# Autodesk Inventor assembly: sheetmetal_cnc
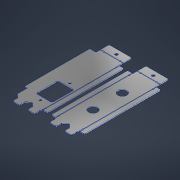
[picture p0: Inventor's stored thumbnail of the model, 180x180]
Saved by Autodesk Inventor 2022 (Build 260153000, 153)
## iProperties
Created: 2025-03-03
Part Number: sheetmetal_cnc
Document SubType Name: Assembly
Designer: gisen
Author: gisen
## Documents named in this file (3)
- C:\Users\gisen\Documents\CAD\inventor\git\eatx_case\eatx_slim\sheetmetal_cnc.iam
- C:\Users\gisen\Documents\CAD\inventor\git\eatx_case\eatx_slim\parts\power_ac_plate.ipt
- C:\Users\gisen\Documents\CAD\inventor\git\eatx_case\eatx_slim\parts\power_sw_plate.ipt
## Components (2 placed, 2 different names)
1. power_ac_plate:1 — フラッシュ:1, フラッシュ:2, メイト:1
2. power_sw_plate:1 — フラッシュ:1, フラッシュ:2, メイト:1
## Relationships (3: Flush 2, Mate 1)
- フラッシュ:1 [Flush]: power_ac_plate:1 ↔ power_sw_plate:1
- フラッシュ:2 [Flush]: power_ac_plate:1 ↔ power_sw_plate:1
- メイト:1 [Mate] (5 mm): power_ac_plate:1 ↔ power_sw_plate:1
